# Autodesk Inventor assembly: POM_T5_11
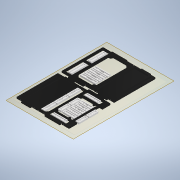
[picture p0: Inventor's stored thumbnail of the model, 180x180]
Saved by Autodesk Inventor 2020.5 (Build 245400000, 400)
## iProperties
Created: 2021-08-27
Part Number: POM_T5_11
Document SubType Name: Assembly
Designer: Masato
Author: Masato
## Documents named in this file (14)
- C:\Users\marin\Documents\0426 git clone\SUSTAINA-OP\Cam\POM_T5_11.iam
- C:\Users\marin\Documents\0426 git clone\SUSTAINA-OP\Cam\DisposableBoard.ipt
- C:\Users\marin\Documents\0426 git clone\SUSTAINA-OP\UpperBody\Cockpit\Cockpit_carrier_board_frame.ipt
- C:\Users\marin\Documents\0426 git clone\SUSTAINA-OP\UpperBody\Cockpit\Cockpit_circuit_board_frame.ipt
- C:\Users\marin\Documents\0426 git clone\SUSTAINA-OP\UpperBody\Cockpit\Cockpit_front_frame.ipt
- C:\Users\marin\Documents\0426 git clone\SUSTAINA-OP\Jig\BackLink_diagonal_Jig.ipt
- C:\Users\marin\Documents\0426 git clone\SUSTAINA-OP\Jig\Shoulder_horn_frame_Jig.ipt
- C:\Users\marin\Documents\0426 git clone\SUSTAINA-OP\Jig\Trunk_chest_frame_Jig_1.ipt
- C:\Users\marin\Documents\0426 git clone\SUSTAINA-OP\Jig\Foot_root_block_Jig.ipt
- C:\Users\marin\Documents\0426 git clone\SUSTAINA-OP\Jig\UpperArm_diagonal_Jig.ipt
- C:\Users\marin\Documents\0426 git clone\SUSTAINA-OP\Jig\FrontLink_diagonal_Jig.ipt
- C:\Users\marin\Documents\0426 git clone\SUSTAINA-OP\Jig\Trunk_lower_side_frame_Jig.ipt
- C:\Users\marin\Documents\0426 git clone\SUSTAINA-OP\Jig\Head_horn_frame_Jig.ipt
- C:\Users\marin\Documents\0426 git clone\SUSTAINA-OP\Jig\Trunk_chest_frame_Jig_2.ipt
## Components (25 placed, 13 different names)
1. DisposableBoard:1 — メイト:2, メイト:1, フラッシュ:1, フラッシュ:2, メイト:5, メイト:9, メイト:12, フラッシュ:3, フラッシュ:4, メイト:13
2. Cockpit_carrier_board_frame:1 — メイト:5, メイト:11, メイト:15, フラッシュ:6, メイト:19, メイト:20, メイト:22, メイト:23, 正接:1, メイト:25, メイト:27, 正接:2, メイト:38, メイト:41, メイト:42
3. Cockpit_circuit_board_frame:1 — メイト:10, フラッシュ:5, メイト:13, メイト:14, メイト:32, メイト:33, メイト:35, メイト:36, 正接:3, メイト:44, メイト:47
4. Cockpit_front_frame:1 — メイト:9, メイト:10, メイト:11
5. Cockpit_front_frame:2 — メイト:12, フラッシュ:3, フラッシュ:4, フラッシュ:5, メイト:14, メイト:15, フラッシュ:6, メイト:39
6. Trunk_chest_frame_Jig_1:2 — メイト:18, メイト:19, メイト:20
7. Trunk_chest_frame_Jig_1:3 — メイト:21, メイト:22, メイト:23
8. FrontLink_diagonal_Jig:1 — メイト:31, メイト:32, メイト:33
9. FrontLink_diagonal_Jig:2 — メイト:34, メイト:35, メイト:36
10. BackLink_diagonal_Jig:6 — メイト:24, 正接:1, メイト:25
11. BackLink_diagonal_Jig:7
12. Shoulder_horn_frame_Jig:1 — メイト:26, メイト:27, 正接:2
13. Shoulder_horn_frame_Jig:2 — メイト:29
14. UpperArm_diagonal_Jig:1 — メイト:28, メイト:29
15. UpperArm_diagonal_Jig:2
16. UpperArm_diagonal_Jig:3
17. Head_horn_frame_Jig:1 — メイト:37, メイト:38, メイト:39
18. Head_horn_frame_Jig:2
19. Head_horn_frame_Jig:3
20. Foot_root_block_Jig:1 — メイト:40, メイト:41, メイト:42
21. Foot_root_block_Jig:2
22. Trunk_chest_frame_Jig_2:1 — メイト:43, 正接:3, メイト:44
23. Trunk_chest_frame_Jig_2:2 — メイト:46
24. Trunk_lower_side_frame_Jig:1 — メイト:45, メイト:46, メイト:47
25. Trunk_lower_side_frame_Jig:2
## Component patterns: (2 elements, first: BackLink_diagonal_Jig:6), (2 elements, first: Shoulder_horn_frame_Jig:1), (3 elements, first: UpperArm_diagonal_Jig:1), (3 elements, first: Head_horn_frame_Jig:1), (2 elements, first: Foot_root_block_Jig:1), (2 elements, first: Trunk_chest_frame_Jig_2:1), (2 elements, first: Trunk_lower_side_frame_Jig:1)
## Relationships (48: Mate 39, Flush 6, Tangent 3)
- メイト:2 [Mate]: DisposableBoard:1
- メイト:1 [Mate]: DisposableBoard:1
- フラッシュ:1 [Flush]: DisposableBoard:1
- フラッシュ:2 [Flush]: DisposableBoard:1
- メイト:5 [Mate]: DisposableBoard:1 ↔ Cockpit_carrier_board_frame:1
- メイト:9 [Mate]: DisposableBoard:1 ↔ Cockpit_front_frame:1
- メイト:10 [Mate] (2.5 mm): Cockpit_circuit_board_frame:1 ↔ Cockpit_front_frame:1
- メイト:11 [Mate] (2.5 mm): Cockpit_carrier_board_frame:1 ↔ Cockpit_front_frame:1
- メイト:12 [Mate]: DisposableBoard:1 ↔ Cockpit_front_frame:2
- フラッシュ:3 [Flush] (2.5 mm): DisposableBoard:1 ↔ Cockpit_front_frame:2
- フラッシュ:4 [Flush] (2.5 mm): DisposableBoard:1 ↔ Cockpit_front_frame:2
- フラッシュ:5 [Flush]: Cockpit_circuit_board_frame:1 ↔ Cockpit_front_frame:2
- メイト:13 [Mate]: DisposableBoard:1 ↔ Cockpit_circuit_board_frame:1
- メイト:14 [Mate] (2.5 mm): Cockpit_circuit_board_frame:1 ↔ Cockpit_front_frame:2
- メイト:15 [Mate] (2.5 mm): Cockpit_carrier_board_frame:1 ↔ Cockpit_front_frame:2
- フラッシュ:6 [Flush]: Cockpit_carrier_board_frame:1 ↔ Cockpit_front_frame:2
- メイト:18 [Mate]: Trunk_chest_frame_Jig_1:2
- メイト:19 [Mate] (2.5 mm): Cockpit_carrier_board_frame:1 ↔ Trunk_chest_frame_Jig_1:2
- メイト:20 [Mate] (6 mm): Cockpit_carrier_board_frame:1 ↔ Trunk_chest_frame_Jig_1:2
- メイト:21 [Mate]: Trunk_chest_frame_Jig_1:3
- メイト:22 [Mate] (2.5 mm): Cockpit_carrier_board_frame:1 ↔ Trunk_chest_frame_Jig_1:3
- メイト:23 [Mate] (6 mm): Cockpit_carrier_board_frame:1 ↔ Trunk_chest_frame_Jig_1:3
- メイト:24 [Mate]: BackLink_diagonal_Jig:6
- 正接:1 [Tangent] (2.5 mm): Cockpit_carrier_board_frame:1 ↔ BackLink_diagonal_Jig:6
- メイト:25 [Mate] (2.5 mm): Cockpit_carrier_board_frame:1 ↔ BackLink_diagonal_Jig:6
- メイト:26 [Mate]: Shoulder_horn_frame_Jig:1
- メイト:27 [Mate] (2.5 mm): Cockpit_carrier_board_frame:1 ↔ Shoulder_horn_frame_Jig:1
- 正接:2 [Tangent] (2.5 mm): Cockpit_carrier_board_frame:1 ↔ Shoulder_horn_frame_Jig:1
- メイト:28 [Mate]: UpperArm_diagonal_Jig:1
- メイト:29 [Mate] (2.5 mm): Shoulder_horn_frame_Jig:2 ↔ UpperArm_diagonal_Jig:1
- メイト:31 [Mate]: FrontLink_diagonal_Jig:1
- メイト:32 [Mate] (4 mm): Cockpit_circuit_board_frame:1 ↔ FrontLink_diagonal_Jig:1
- メイト:33 [Mate] (5 mm): Cockpit_circuit_board_frame:1 ↔ FrontLink_diagonal_Jig:1
- メイト:34 [Mate]: FrontLink_diagonal_Jig:2
- メイト:35 [Mate] (4 mm): Cockpit_circuit_board_frame:1 ↔ FrontLink_diagonal_Jig:2
- メイト:36 [Mate] (5 mm): Cockpit_circuit_board_frame:1 ↔ FrontLink_diagonal_Jig:2
- メイト:37 [Mate]: Head_horn_frame_Jig:1
- メイト:38 [Mate] (2.5 mm): Cockpit_carrier_board_frame:1 ↔ Head_horn_frame_Jig:1
- メイト:39 [Mate] (5 mm): Cockpit_front_frame:2 ↔ Head_horn_frame_Jig:1
- メイト:40 [Mate]: Foot_root_block_Jig:1
- メイト:41 [Mate] (2.5 mm): Cockpit_carrier_board_frame:1 ↔ Foot_root_block_Jig:1
- メイト:42 [Mate] (2.5 mm): Cockpit_carrier_board_frame:1 ↔ Foot_root_block_Jig:1
- メイト:43 [Mate]: Trunk_chest_frame_Jig_2:1
- 正接:3 [Tangent] (2.5 mm): Cockpit_circuit_board_frame:1 ↔ Trunk_chest_frame_Jig_2:1
- メイト:44 [Mate] (7 mm): Cockpit_circuit_board_frame:1 ↔ Trunk_chest_frame_Jig_2:1
- メイト:45 [Mate]: Trunk_lower_side_frame_Jig:1
- メイト:46 [Mate] (2.5 mm): Trunk_chest_frame_Jig_2:2 ↔ Trunk_lower_side_frame_Jig:1
- メイト:47 [Mate] (8 mm): Cockpit_circuit_board_frame:1 ↔ Trunk_lower_side_frame_Jig:1
